# Autodesk Inventor assembly: hole reference
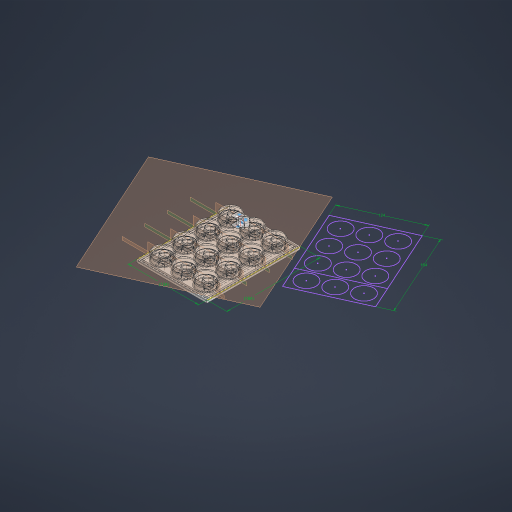
[picture p0: Inventor's stored thumbnail of the model, 512x512]
Saved by Autodesk Inventor 2023 (Build 270158030, 158C)
## iProperties
Created: 2022-06-20
Part Number: hole reference
Document SubType Name: Assembly
Designer: Simon
Author: Simon
## Documents named in this file (3)
- C:\Users\simfe\Desktop\2.Semester\Technische Grundlagen-II\Pixie\3d-modelle\.iam's\hole reference.iam
- C:\Users\simfe\Desktop\2.Semester\Technische Grundlagen-II\Pixie\3d-modelle\.ipt's\Groundplate.ipt
- C:\Users\simfe\Desktop\2.Semester\Technische Grundlagen-II\Pixie\3d-modelle\.ipt's\Button adapter.ipt
## Components (13 placed, 2 different names)
1. Groundplate:1 — Mate:10, Mate:11, Mate:12
2. Button adapter:4 — Mate:10, Mate:11, Mate:12, Flush:1
3. Button adapter:5
4. Button adapter:6
5. Button adapter:7
6. Button adapter:8
7. Button adapter:9
8. Button adapter:10
9. Button adapter:11
10. Button adapter:12
11. Button adapter:13
12. Button adapter:14
13. Button adapter:15
## Component patterns: (12 elements, first: Button adapter:4)
## Relationships (4: Mate 3, Flush 1)
- Mate:10: Groundplate:1 ↔ Button adapter:4
- Mate:11: Groundplate:1 ↔ Button adapter:4
- Mate:12: Groundplate:1 ↔ Button adapter:4
- Flush:1 (10.25 mm): Button adapter:4
